# Autodesk Inventor assembly: Body
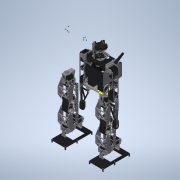
[picture p0: Inventor's stored thumbnail of the model, 180x180]
Saved by Autodesk Inventor 2020.4 (Build 244396000, 396)
## iProperties
Created: 2021-09-30
Part Number: Body
Document SubType Name: Assembly
Designer: Masato Kubotera
Mass: 4463.19 g
Surface Area: 13321.9 cm^2
Volume: 2213.37 cm^3
Density: 2.01647 g/cm^3
Author: Masato Kubotera
## Documents named in this file (3)
- C:\Users\Masato\Documents\Inventor\CIT Brains_Inventor\OpenPlatform_ver3_0 - ve4_1 branch\Body.iam
- C:\Users\Masato\Documents\Inventor\CIT Brains_Inventor\OpenPlatform_ver3_0 - ve4_1 branch\UpperBody\UpperBody.iam
- C:\Users\Masato\Documents\Inventor\CIT Brains_Inventor\OpenPlatform_ver3_0 - ve4_1 branch\LowerBody\LowerBody.iam
## Components (3 placed, 2 different names)
1. UpperBody:1 [sub-assembly] — 挿入:3, 角度:2
2. LowerBody:1 [sub-assembly] — 挿入:3, 角度:2
3. LowerBody:2 [sub-assembly]
## Relationships (2: Insert 1, Angle 1)
- 挿入:3 [Insert]: UpperBody:1 ↔ LowerBody:1
- 角度:2 [Angle] (0 deg): UpperBody:1 ↔ LowerBody:1
